# Autodesk Inventor assembly: engine assembly
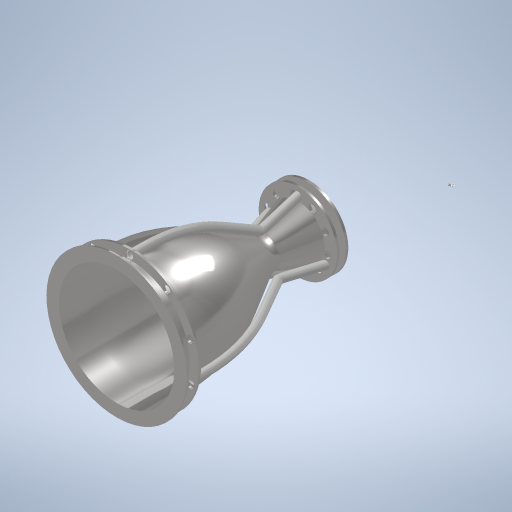
[picture p0: Inventor's stored thumbnail of the model, 512x512]
Saved by Autodesk Inventor 2023 (Build 270158000, 158)
## iProperties
Created: 2022-07-21
Part Number: engine assembly
Document SubType Name: Assembly
Designer: station
Mass: 3659.88 g
Surface Area: 4755.26 cm^2
Volume: 455.583 cm^3
Density: 8.0334 g/cm^3
Author: station
## Documents named in this file (8)
- C:\Users\station\Documents\Project\Liquid-engine-cooling-system\design files\Ethanol engine 5 -inventor\engine assembly.iam
- C:\Users\station\Documents\Project\Liquid-engine-cooling-system\design files\Ethanol engine 5 -inventor\inner wall.ipt
- C:\Users\station\Documents\Project\Liquid-engine-cooling-system\design files\Ethanol engine 5 -inventor\new outer wall.ipt
- C:\Users\station\Documents\Project\Liquid-engine-cooling-system\design files\Ethanol engine 5 -inventor\back bracket 2.ipt
- C:\Users\station\Documents\Project\Liquid-engine-cooling-system\design files\Ethanol engine 5 -inventor\back bracket.ipt
- C:\Users\station\Documents\Project\Liquid-engine-cooling-system\design files\Ethanol engine 5 -inventor\bracket 1.ipt
- C:\Users\station\Documents\Project\Liquid-engine-cooling-system\design files\Ethanol engine 5 -inventor\temperature sensor.ipt
- C:\Users\station\Documents\Project\Liquid-engine-cooling-system\design files\Ethanol engine 5 -inventor\ethanol engine 5 v7.iam
## Components (10 placed, 7 different names)
1. inner wall:1 — Mate:1, Flush:1, Mate:2, Mate:4
2. new outer wall:1 — Mate:1, Flush:1, Mate:3, Mate:5, Mate:6, Mate:7
3. back bracket 2:1 — Mate:2, Mate:3, Mate:8
4. back bracket:1 — Mate:4, Mate:5, Mate:8
5. bracket 1:1 — Mate:6, Mate:7
6. temperature sensor:1
7. ethanol engine 5 v7:1 [sub-assembly]
8. ethanol engine 5 v7:2 [sub-assembly]
9. ethanol engine 5 v7:3 [sub-assembly]
10. ethanol engine 5 v7:4 [sub-assembly]
## Relationships (9: Mate 8, Flush 1)
- Mate:1: inner wall:1 ↔ new outer wall:1
- Flush:1: inner wall:1 ↔ new outer wall:1
- Mate:2: inner wall:1 ↔ back bracket 2:1
- Mate:3 (-14.601 mm): new outer wall:1 ↔ back bracket 2:1
- Mate:4: inner wall:1 ↔ back bracket:1
- Mate:5 (-3.601 mm): new outer wall:1 ↔ back bracket:1
- Mate:6: new outer wall:1 ↔ bracket 1:1
- Mate:7 (-18 mm): new outer wall:1 ↔ bracket 1:1
- Mate:8: back bracket 2:1 ↔ back bracket:1
